# Autodesk Inventor assembly: cellSTORM_v5_Alvium_dualcolour
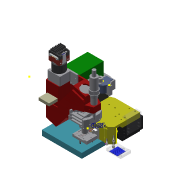
[picture p0: Inventor's stored thumbnail of the model, 180x180]
Saved by Autodesk Inventor 2019.4 (Build 234330000, 330)
## iProperties
Created: 2020-04-25
Part Number: cellSTORM_v5_Alvium_dualcolour
Document SubType Name: Assembly
Designer: diederichbenedict
Author: diederichbenedict
## Documents named in this file (35)
- C:\Users\diederichbenedict\Dropbox\Dokumente\Promotion\PROJECTS\STORMoChip\GITHUB\CAD\Nanoscopy-on-the-cheap\Workspace\cellSTORM_v5_Alvium_dualcolour.iam
- C:\Users\diederichbenedict\Dropbox\Dokumente\Promotion\PROJECTS\STORMoChip\GITHUB\CAD\Nanoscopy-on-the-cheap\Workspace\00_LASER_640nm.ipt
- C:\Users\diederichbenedict\Dropbox\Dokumente\Promotion\PROJECTS\STORMoChip\GITHUB\CAD\Nanoscopy-on-the-cheap\Workspace\00_XY_stage-CHUO_SEIKI_LD-647-R1.iam
- C:\Users\diederichbenedict\Dropbox\Dokumente\Promotion\PROJECTS\STORMoChip\GITHUB\CAD\Nanoscopy-on-the-cheap\Workspace\02_Nanoscopy_Chip.ipt
- C:\Users\diederichbenedict\Dropbox\Dokumente\Promotion\PROJECTS\STORMoChip\GITHUB\CAD\Nanoscopy-on-the-cheap\Workspace\00_Ballmagnets_5mm.ipt
- C:\Users\diederichbenedict\Documents\Inventor\Content Center Files\R2019\en-US\DIN 912\DIN 912 - M3 x 0.5 x 25 x 18.ipt
- C:\Users\diederichbenedict\Dropbox\Dokumente\Promotion\PROJECTS\STORMoChip\GITHUB\CAD\Nanoscopy-on-the-cheap\Workspace\cellSTORM_Base_v0_R1.ipt
- C:\Users\diederichbenedict\Dropbox\Dokumente\Promotion\PROJECTS\STORMoChip\GITHUB\CAD\Nanoscopy-on-the-cheap\Workspace\00_KES400.iam
- C:\Users\diederichbenedict\Dropbox\Dokumente\Promotion\PROJECTS\STORMoChip\GITHUB\CAD\Nanoscopy-on-the-cheap\Workspace\cellSTORM_v5_cellphonestage.ipt
- C:\Users\diederichbenedict\Dropbox\Dokumente\Promotion\PROJECTS\STORMoChip\GITHUB\CAD\Nanoscopy-on-the-cheap\Workspace\cellSTORM_v5_microscope_cover.ipt
- C:\Users\diederichbenedict\Dropbox\Dokumente\Promotion\PROJECTS\STORMoChip\GITHUB\CAD\Nanoscopy-on-the-cheap\Workspace\00_Stepper_Motor_28BYJ-48.0013.ipt
- C:\Users\diederichbenedict\Dropbox\Dokumente\Promotion\PROJECTS\STORMoChip\GITHUB\CAD\Nanoscopy-on-the-cheap\Workspace\cellSTORM_v5_focusmotormount.ipt
- C:\Users\diederichbenedict\Dropbox\Dokumente\Promotion\PROJECTS\STORMoChip\GITHUB\CAD\Nanoscopy-on-the-cheap\Workspace\BD-DRIVE_PULLEY.ipt
- C:\Users\diederichbenedict\Dropbox\Dokumente\Promotion\PROJECTS\STORMoChip\GITHUB\CAD\Nanoscopy-on-the-cheap\Workspace\cellSTORM_focusmotor_pulley.ipt
- C:\Users\diederichbenedict\Dropbox\Dokumente\Promotion\PROJECTS\STORMoChip\GITHUB\CAD\Nanoscopy-on-the-cheap\Workspace\cellSTORM_v5_ELECTRONICS.iam
- C:\Users\diederichbenedict\Dropbox\Dokumente\Promotion\PROJECTS\STORMoChip\GITHUB\CAD\Nanoscopy-on-the-cheap\Workspace\00_chip_01_old.ipt
- C:\Users\diederichbenedict\Dropbox\Dokumente\Promotion\PROJECTS\STORMoChip\GITHUB\CAD\Nanoscopy-on-the-cheap\Workspace\cellSTORM_v5_chiptray_old_0.ipt
- C:\Users\diederichbenedict\Dropbox\Dokumente\Promotion\PROJECTS\STORMoChip\GITHUB\CAD\Nanoscopy-on-the-cheap\Workspace\cellSTORM_v5_chiptry_clamp.ipt
- C:\Users\diederichbenedict\Dropbox\Dokumente\Promotion\PROJECTS\STORMoChip\GITHUB\CAD\Nanoscopy-on-the-cheap\Workspace\00_chip_01_new.ipt
- C:\Users\diederichbenedict\Dropbox\Dokumente\Promotion\PROJECTS\STORMoChip\GITHUB\CAD\Nanoscopy-on-the-cheap\Workspace\cellSTORM_v5_chiptray_new_0.ipt
- C:\Users\diederichbenedict\Dropbox\Dokumente\Promotion\PROJECTS\STORMoChip\GITHUB\CAD\Nanoscopy-on-the-cheap\Workspace\00_Laser_532nm_200mw.ipt
- C:\Users\diederichbenedict\Dropbox\Dokumente\Promotion\PROJECTS\STORMoChip\GITHUB\CAD\Nanoscopy-on-the-cheap\Workspace\cellSTORM_v5_cellphonespacer.ipt
- C:\Users\diederichbenedict\Dropbox\Dokumente\Promotion\PROJECTS\STORMoChip\GITHUB\CAD\Nanoscopy-on-the-cheap\Workspace\cellSTORM_v5_laserstage_dualcolour.ipt
- C:\Users\diederichbenedict\Dropbox\Dokumente\Promotion\PROJECTS\STORMoChip\GITHUB\CAD\Nanoscopy-on-the-cheap\Workspace\cellSTORM_laserbeam_dual.ipt
- C:\Users\diederichbenedict\Dropbox\Dokumente\Promotion\PROJECTS\STORMoChip\GITHUB\CAD\Nanoscopy-on-the-cheap\Workspace\00_KES400_DichroicMirror.ipt
- C:\Users\diederichbenedict\Dropbox\Dokumente\Promotion\PROJECTS\STORMoChip\GITHUB\CAD\Nanoscopy-on-the-cheap\Workspace\00_ComarMirror_10mm.ipt
- C:\Users\diederichbenedict\Dropbox\Dokumente\Promotion\PROJECTS\STORMoChip\GITHUB\CAD\Nanoscopy-on-the-cheap\Workspace\cellSTORM_v5_beamaligner.ipt
- C:\Users\diederichbenedict\Dropbox\Dokumente\Promotion\PROJECTS\STORMoChip\GITHUB\CAD\Nanoscopy-on-the-cheap\Workspace\cellSTORM_v5_microsocpe_alliedvision.iam
- C:\Users\diederichbenedict\Dropbox\Dokumente\Promotion\PROJECTS\STORMoChip\GITHUB\CAD\Nanoscopy-on-the-cheap\Workspace\cellSTORM_v5_spacer_xy_stage.ipt
- C:\Users\diederichbenedict\Dropbox\Dokumente\Promotion\PROJECTS\STORMoChip\GITHUB\CAD\Nanoscopy-on-the-cheap\Workspace\00_COMAR_521_IY_16.ipt
- C:\Users\diederichbenedict\Dropbox\Dokumente\Promotion\PROJECTS\STORMoChip\GITHUB\CAD\Nanoscopy-on-the-cheap\Workspace\cellSTORM_dichroic_mirror_adjuster_comar_16mm.ipt
- C:\Users\diederichbenedict\Dropbox\Dokumente\Promotion\PROJECTS\STORMoChip\GITHUB\CAD\Nanoscopy-on-the-cheap\Workspace\cellSTORM_Laserrotator_v0.ipt
- C:\Users\diederichbenedict\Dropbox\Dokumente\Promotion\PROJECTS\STORMoChip\GITHUB\CAD\Nanoscopy-on-the-cheap\Workspace\cellSTORM_v5_chiptray_adjustmentscrew.ipt
- C:\Users\diederichbenedict\Dropbox\Dokumente\Promotion\PROJECTS\STORMoChip\GITHUB\CAD\Nanoscopy-on-the-cheap\Workspace\00_microscope_slide.ipt
- C:\Users\diederichbenedict\Dropbox\Dokumente\Promotion\PROJECTS\STORMoChip\GITHUB\CAD\Nanoscopy-on-the-cheap\Workspace\cellSTORM_v5_chiptray_brightfieldslide.ipt
## Components (44 placed, 34 different names)
1. 00_LASER_640nm:1 — Insert:2, Angle:6, Mate:7, Mate:6, Flush:1, Angle:7
2. 00_XY_stage-CHUO_SEIKI_LD-647-R1:1 [sub-assembly] — Insert:1, Angle:1, Insert:6, Angle:5, Mate:6, Flush:1, Flush:10, Flush:11, Flush:41
3. cellSTORM_laserbeam_dual:1 — Insert:2, Insert:3, Insert:7, Insert:16, Mate:27, Mate:28, Angle:9, Tangent:1, Angle:10, Mate:29, Flush:35, Mate:30, Mate:31, Insert:17, Tangent:3, Mate:32
4. 02_Nanoscopy_Chip:1 — Insert:3, Angle:2, Mate:11
5. 00_Ballmagnets_5mm:1
6. DIN 912 - replaced by DIN EN ISO 4762 M3 x 25:1 — Insert:4, Flush:35
7. 00_Ballmagnets_5mm:2
8. DIN 912 - replaced by DIN EN ISO 4762 M3 x 25:2 — Insert:13
9. 00_Ballmagnets_5mm:3
10. DIN 912 - replaced by DIN EN ISO 4762 M3 x 25:3 — Insert:14
11. cellSTORM_Base_v0_R1:1 — Insert:1, Angle:1, Angle:2, Insert:4, Angle:6, Mate:7, Insert:13, Insert:14, Flush:23
12. 00_XY_stage-CHUO_SEIKI_LD-647-R1:2 [sub-assembly] — Insert:6, Angle:5, Flush:12, Flush:13, Flush:32
13. 00_KES400:1 [sub-assembly] — Insert:7, Angle:7, Mate:27
14. cellSTORM_v5_laserstage_dualcolour:1 — Flush:10, Flush:11, Flush:33, Angle:8, Flush:36, Flush:37, Flush:38, Insert:18, Insert:19, Insert:20, Flush:39, Flush:42, Flush:43
15. cellSTORM_v5_cellphonestage:1 — Flush:12, Flush:13, Mate:10, Flush:14, Flush:17, Flush:18, Flush:19
16. cellSTORM_v5_microsocpe_alliedvision:1 [sub-assembly] — Mate:10, Mate:11, Flush:14, Flush:15, Flush:16, Mate:18, Mate:19, Mate:20, Insert:21
17. cellSTORM_v5_microscope_cover:1 — Flush:15, Flush:16
18. 00_Stepper_Motor_28BYJ-48.0013:1 — Mate:18, Mate:19, Flush:17, Flush:20, Insert:15
19. cellSTORM_v5_focusmotormount:1 — Flush:18, Flush:19, Flush:20, Flush:31
20. BD-DRIVE_PULLEY:1 — Insert:15, Flush:21
21. cellSTORM_focusmotor_pulley:1 — Mate:20, Flush:21, Insert:21
22. cellSTORM_v5_ELECTRONICS:1 [sub-assembly]
23. 00_chip_01_old:1 — Flush:22, Insert:16
24. cellSTORM_v5_chiptray_old_0:1 — Flush:22, Flush:23, Flush:24, Flush:25, Flush:44, Flush:45
25. cellSTORM_v5_chiptry_clamp:1 — Flush:24, Flush:25
26. 00_chip_01_new:1 — Mate:25, Mate:26, Flush:26
27. cellSTORM_v5_chiptray_new_0:1 — Mate:25, Mate:26, Flush:26
28. cellSTORM_v5_cellphonespacer:1 — Flush:31, Flush:32
29. 00_Laser_532nm_200mw:3 — Mate:28, Flush:33, Angle:8, Tangent:2, Flush:34
30. 00_LASER_640nm:2 — Mate:29, Flush:34
31. 00_KES400_DichroicMirror:1 — Mate:30, Mate:31, Angle:11
32. 00_ComarMirror_10mm:1 — Insert:17, Flush:36
33. cellSTORM_v5_beamaligner:1 — Flush:37, Flush:38
34. DIN 912 - replaced by DIN EN ISO 4762 M3 x 25:4 — Insert:18
35. DIN 912 - replaced by DIN EN ISO 4762 M3 x 25:5 — Insert:19
36. DIN 912 - replaced by DIN EN ISO 4762 M3 x 25:6 — Insert:20
37. cellSTORM_dichroic_mirror_adjuster_comar_16mm:2 — Flush:39
38. cellSTORM_v5_spacer_xy_stage:1 — Flush:41
39. 00_COMAR_521_IY_16:1 — Mate:32
40. cellSTORM_dichroic_mirror_adjuster_comar_16mm:1
41. cellSTORM_Laserrotator_v0:1 — Flush:42, Flush:43
42. cellSTORM_v5_chiptray_adjustmentscrew:1 — Flush:44, Flush:45
43. 00_microscope_slide:1
44. cellSTORM_v5_chiptray_brightfieldslide:1
## Relationships (77: Flush 32, Mate 18, Insert 15, Angle 9, Tangent 3)
- [Mate]: 00_Ballmagnets_5mm:1 ↔ DIN 912 - replaced by DIN EN ISO 4762 M3 x 25:1
- [Mate]: 00_Ballmagnets_5mm:2 ↔ DIN 912 - replaced by DIN EN ISO 4762 M3 x 25:2
- [Mate]: 00_Ballmagnets_5mm:3 ↔ DIN 912 - replaced by DIN EN ISO 4762 M3 x 25:3
- Insert:1: 00_XY_stage-CHUO_SEIKI_LD-647-R1:1 ↔ cellSTORM_Base_v0_R1:1
- Angle:1 (90 deg): 00_XY_stage-CHUO_SEIKI_LD-647-R1:1 ↔ cellSTORM_Base_v0_R1:1
- Insert:2 (-10 mm): 00_LASER_640nm:1 ↔ cellSTORM_laserbeam_dual:1
- Insert:3 (5 mm): cellSTORM_laserbeam_dual:1 ↔ 02_Nanoscopy_Chip:1
- Angle:2 (180 deg): 02_Nanoscopy_Chip:1 ↔ cellSTORM_Base_v0_R1:1
- Insert:4 (-15 mm): DIN 912 - replaced by DIN EN ISO 4762 M3 x 25:1 ↔ cellSTORM_Base_v0_R1:1
- Insert:6 (6 mm): 00_XY_stage-CHUO_SEIKI_LD-647-R1:1 ↔ 00_XY_stage-CHUO_SEIKI_LD-647-R1:2
- Angle:5 (180 deg): 00_XY_stage-CHUO_SEIKI_LD-647-R1:1 ↔ 00_XY_stage-CHUO_SEIKI_LD-647-R1:2
- Angle:6 (0 deg): 00_LASER_640nm:1 ↔ cellSTORM_Base_v0_R1:1
- Mate:7 (1 mm): 00_LASER_640nm:1 ↔ cellSTORM_Base_v0_R1:1
- Mate:6 (10 mm): 00_LASER_640nm:1 ↔ 00_XY_stage-CHUO_SEIKI_LD-647-R1:1
- Flush:1 (-5 mm): 00_LASER_640nm:1 ↔ 00_XY_stage-CHUO_SEIKI_LD-647-R1:1
- Insert:7: cellSTORM_laserbeam_dual:1 ↔ 00_KES400:1
- Angle:7 (0 deg): 00_LASER_640nm:1 ↔ 00_KES400:1
- Insert:13 (-15 mm): DIN 912 - replaced by DIN EN ISO 4762 M3 x 25:2 ↔ cellSTORM_Base_v0_R1:1
- Insert:14 (-15 mm): DIN 912 - replaced by DIN EN ISO 4762 M3 x 25:3 ↔ cellSTORM_Base_v0_R1:1
- Flush:10: 00_XY_stage-CHUO_SEIKI_LD-647-R1:1 ↔ cellSTORM_v5_laserstage_dualcolour:1
- Flush:11: 00_XY_stage-CHUO_SEIKI_LD-647-R1:1 ↔ cellSTORM_v5_laserstage_dualcolour:1
- Flush:12: 00_XY_stage-CHUO_SEIKI_LD-647-R1:2 ↔ cellSTORM_v5_cellphonestage:1
- Flush:13: 00_XY_stage-CHUO_SEIKI_LD-647-R1:2 ↔ cellSTORM_v5_cellphonestage:1
- Mate:10: cellSTORM_v5_cellphonestage:1 ↔ cellSTORM_v5_microsocpe_alliedvision:1
- Mate:11: 02_Nanoscopy_Chip:1 ↔ cellSTORM_v5_microsocpe_alliedvision:1
- Flush:14: cellSTORM_v5_cellphonestage:1 ↔ cellSTORM_v5_microsocpe_alliedvision:1
- Flush:15: cellSTORM_v5_microsocpe_alliedvision:1 ↔ cellSTORM_v5_microscope_cover:1
- Flush:16: cellSTORM_v5_microsocpe_alliedvision:1 ↔ cellSTORM_v5_microscope_cover:1
- Mate:18 (10 mm): cellSTORM_v5_microsocpe_alliedvision:1 ↔ 00_Stepper_Motor_28BYJ-48.0013:1
- Mate:19 (35 mm): cellSTORM_v5_microsocpe_alliedvision:1 ↔ 00_Stepper_Motor_28BYJ-48.0013:1
- Flush:17 (-40 mm): cellSTORM_v5_cellphonestage:1 ↔ 00_Stepper_Motor_28BYJ-48.0013:1
- Flush:18: cellSTORM_v5_cellphonestage:1 ↔ cellSTORM_v5_focusmotormount:1
- Flush:19: cellSTORM_v5_cellphonestage:1 ↔ cellSTORM_v5_focusmotormount:1
- Flush:20: 00_Stepper_Motor_28BYJ-48.0013:1 ↔ cellSTORM_v5_focusmotormount:1
- Insert:15: 00_Stepper_Motor_28BYJ-48.0013:1 ↔ BD-DRIVE_PULLEY:1
- Mate:20: cellSTORM_v5_microsocpe_alliedvision:1 ↔ cellSTORM_focusmotor_pulley:1
- Flush:21: BD-DRIVE_PULLEY:1 ↔ cellSTORM_focusmotor_pulley:1
- Flush:22: 00_chip_01_old:1 ↔ cellSTORM_v5_chiptray_old_0:1
- Flush:23 (10 mm): cellSTORM_Base_v0_R1:1 ↔ cellSTORM_v5_chiptray_old_0:1
- Insert:16: cellSTORM_laserbeam_dual:1 ↔ 00_chip_01_old:1
- Flush:24: cellSTORM_v5_chiptray_old_0:1 ↔ cellSTORM_v5_chiptry_clamp:1
- Flush:25: cellSTORM_v5_chiptray_old_0:1 ↔ cellSTORM_v5_chiptry_clamp:1
- Mate:25: 00_chip_01_new:1 ↔ cellSTORM_v5_chiptray_new_0:1
- Mate:26: 00_chip_01_new:1 ↔ cellSTORM_v5_chiptray_new_0:1
- Flush:26 (-3 mm): 00_chip_01_new:1 ↔ cellSTORM_v5_chiptray_new_0:1
- Mate:27: cellSTORM_laserbeam_dual:1 ↔ 00_KES400:1
- Flush:31: cellSTORM_v5_focusmotormount:1 ↔ cellSTORM_v5_cellphonespacer:1
- Flush:32: 00_XY_stage-CHUO_SEIKI_LD-647-R1:2 ↔ cellSTORM_v5_cellphonespacer:1
- Mate:28: cellSTORM_laserbeam_dual:1 ↔ 00_Laser_532nm_200mw:3
- Flush:33 (-10 mm): cellSTORM_v5_laserstage_dualcolour:1 ↔ 00_Laser_532nm_200mw:3
- Angle:8 (0 deg): cellSTORM_v5_laserstage_dualcolour:1 ↔ 00_Laser_532nm_200mw:3
- Angle:9 (0 deg): cellSTORM_laserbeam_dual:1
- Tangent:1: cellSTORM_laserbeam_dual:1
- Angle:10 (0 deg): cellSTORM_laserbeam_dual:1
- Tangent:2: 00_Laser_532nm_200mw:3
- Mate:29: cellSTORM_laserbeam_dual:1 ↔ 00_LASER_640nm:2
- Flush:34: 00_Laser_532nm_200mw:3 ↔ 00_LASER_640nm:2
- Flush:35: cellSTORM_laserbeam_dual:1 ↔ DIN 912 - replaced by DIN EN ISO 4762 M3 x 25:1
- Mate:30: cellSTORM_laserbeam_dual:1 ↔ 00_KES400_DichroicMirror:1
- Mate:31: cellSTORM_laserbeam_dual:1 ↔ 00_KES400_DichroicMirror:1
- Insert:17: cellSTORM_laserbeam_dual:1 ↔ 00_ComarMirror_10mm:1
- Flush:36: cellSTORM_v5_laserstage_dualcolour:1 ↔ 00_ComarMirror_10mm:1
- Flush:37: cellSTORM_v5_laserstage_dualcolour:1 ↔ cellSTORM_v5_beamaligner:1
- Flush:38: cellSTORM_v5_laserstage_dualcolour:1 ↔ cellSTORM_v5_beamaligner:1
- Insert:18 (-10 mm): cellSTORM_v5_laserstage_dualcolour:1 ↔ DIN 912 - replaced by DIN EN ISO 4762 M3 x 25:4
- Insert:19 (-10 mm): cellSTORM_v5_laserstage_dualcolour:1 ↔ DIN 912 - replaced by DIN EN ISO 4762 M3 x 25:5
- Insert:20 (-10 mm): cellSTORM_v5_laserstage_dualcolour:1 ↔ DIN 912 - replaced by DIN EN ISO 4762 M3 x 25:6
- Flush:39: cellSTORM_v5_laserstage_dualcolour:1 ↔ cellSTORM_dichroic_mirror_adjuster_comar_16mm:2
- Flush:41: 00_XY_stage-CHUO_SEIKI_LD-647-R1:1 ↔ cellSTORM_v5_spacer_xy_stage:1
- Angle:11 (0 deg): 00_KES400_DichroicMirror:1
- Tangent:3: cellSTORM_laserbeam_dual:1
- Mate:32: cellSTORM_laserbeam_dual:1 ↔ 00_COMAR_521_IY_16:1
- Flush:42: cellSTORM_v5_laserstage_dualcolour:1 ↔ cellSTORM_Laserrotator_v0:1
- Flush:43: cellSTORM_v5_laserstage_dualcolour:1 ↔ cellSTORM_Laserrotator_v0:1
- Flush:44: cellSTORM_v5_chiptray_old_0:1 ↔ cellSTORM_v5_chiptray_adjustmentscrew:1
- Flush:45: cellSTORM_v5_chiptray_old_0:1 ↔ cellSTORM_v5_chiptray_adjustmentscrew:1
- Insert:21 (30 mm): cellSTORM_v5_microsocpe_alliedvision:1 ↔ cellSTORM_focusmotor_pulley:1
## Named parameters: d2_d162 = 0 mm, d3_d162 = 0 mm
